# Autodesk Inventor assembly: Enclosure
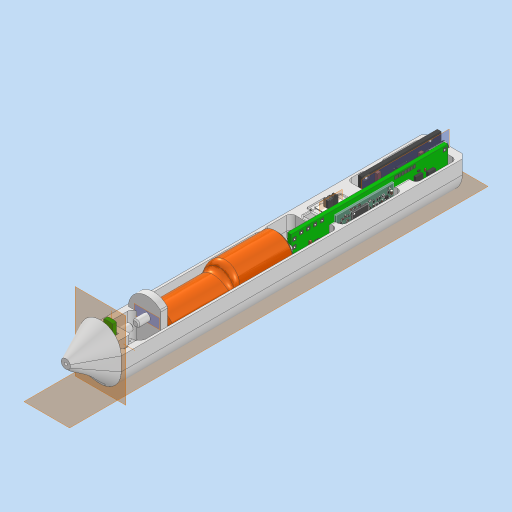
[picture p0: Inventor's stored thumbnail of the model, 512x512]
Saved by Autodesk Inventor 2024 (Build 280153000, 153)
## iProperties
Created: 2025-02-15
Part Number: Enclosure
Document SubType Name: Assembly
Designer: XxPan
Author: XxPan
## Documents named in this file (8)
- C:\Users\XxPan\OneDrive - McMaster University\4OI6\InkSync\case\Enclosure.iam
- C:\Users\XxPan\OneDrive - McMaster University\4OI6\InkSync\case\MCU_PCB.iam
- C:\Users\XxPan\OneDrive - McMaster University\4OI6\InkSync\case\Sensor_PCB.iam
- C:\Users\XxPan\OneDrive - McMaster University\4OI6\InkSync\case\Battery.ipt
- C:\Users\XxPan\OneDrive - McMaster University\4OI6\InkSync\case\Charging_board.ipt
- C:\Users\XxPan\OneDrive - McMaster University\4OI6\InkSync\case\Shell.ipt
- C:\Users\XxPan\OneDrive - McMaster University\4OI6\InkSync\case\Power_switch.ipt
- C:\Users\XxPan\OneDrive - McMaster University\4OI6\InkSync\case\Spring_pin.ipt
## Components (7 placed, 7 different names)
1. MCU_PCB:1 [sub-assembly] — Flush:13, Mate:5, Mate:6
2. Sensor_PCB:1 [sub-assembly] — Flush:5, Flush:6, Flush:7, Flush:8, Flush:11
3. Battery:1 — Angle:1, Insert:2
4. Charging_board:1 — Flush:12, Mate:3, Mate:4, Flush:13, Mate:5, Mate:6
5. Shell:1 — Flush:11, Flush:12, Mate:4, Insert:1, Angle:1, Insert:2
6. Power_switch:1 — Flush:15, Flush:14, Flush:16
7. Spring_pin:1 — Insert:1
## Relationships (17: Flush 10, Mate 4, Insert 2, Angle 1)
- Flush:5: Sensor_PCB:1
- Flush:6: Sensor_PCB:1
- Flush:7: Sensor_PCB:1
- Flush:8: Sensor_PCB:1
- Flush:11 (12 mm): Sensor_PCB:1 ↔ Shell:1
- Flush:12 (0.5 mm): Charging_board:1 ↔ Shell:1
- Mate:3: Charging_board:1
- Mate:4: Charging_board:1 ↔ Shell:1
- Flush:13 (3 mm): MCU_PCB:1 ↔ Charging_board:1
- Mate:5 (1 mm): MCU_PCB:1 ↔ Charging_board:1
- Mate:6: MCU_PCB:1 ↔ Charging_board:1
- Flush:15: Power_switch:1
- Flush:14: Power_switch:1
- Flush:16 (-95 mm): Power_switch:1
- Insert:1: Shell:1 ↔ Spring_pin:1
- Angle:1 (180 deg): Battery:1 ↔ Shell:1
- Insert:2 (-25 mm): Battery:1 ↔ Shell:1
